# Autodesk Inventor assembly: ЕТЗ
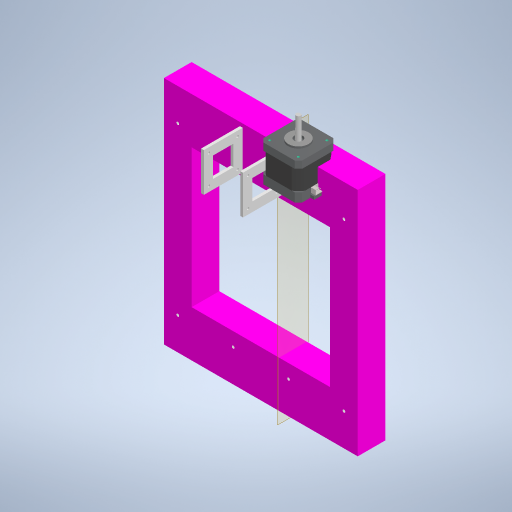
[picture p0: Inventor's stored thumbnail of the model, 512x512]
Saved by Autodesk Inventor 2024.2 (Build 282272000, 272)
## iProperties
Created: 2025-11-19
Part Number: ЕТЗ
Document SubType Name: Assembly
Designer: Zakhar
Author: Zakhar
## Documents named in this file (3)
- C:\Users\Zakhar\Documents\Деталь ВсОШ\ЕТЗ.iam
- C:\Users\Zakhar\Documents\Деталь ВсОШ\ОСНОВА.ipt
- C:\Users\Zakhar\Documents\Деталь ВсОШ\NEMA17 42-40.ipt
## Components (2 placed, 2 different names)
1. ОСНОВА:1 — Жесткий:1
2. NEMA17 42-40:1 — Жесткий:1
## Relationships (1: WeldJoint 1)
- Жесткий:1 [WeldJoint]: ОСНОВА:1 ↔ NEMA17 42-40:1
